# Autodesk Inventor assembly: CaseC
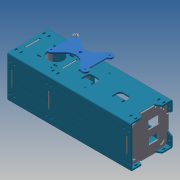
[picture p0: Inventor's stored thumbnail of the model, 180x180]
Saved by Autodesk Inventor 2017 (Build 210142000, 142)
## iProperties
Part Number: CaseC
Material: Genérico
Document SubType Name: Assembly
Designer: Leo
Author: Leo
## Documents named in this file (7)
- C:\Users\FABLAB\Documents\GitHub\actor-re-actor\models\inventor-caja\Case\CaseC.iam
- C:\Users\FABLAB\Documents\GitHub\actor-re-actor\models\inventor-caja\Case\Protector.ipt
- C:\Users\FABLAB\Documents\GitHub\actor-re-actor\models\inventor-caja\Case\Pieza4.ipt
- C:\Users\FABLAB\Documents\GitHub\actor-re-actor\models\inventor-caja\Case\Pliegue Principal.ipt
- C:\Users\FABLAB\Documents\GitHub\actor-re-actor\models\inventor-caja\Case\refuerzo interior.ipt
- C:\Users\FABLAB\Documents\GitHub\actor-re-actor\models\inventor-caja\Case\Tapa Enchufes b.ipt
- C:\Users\FABLAB\Documents\GitHub\actor-re-actor\models\inventor-caja\Case\CaseC\Design Accelerator\Conexión por perno1.iam
## Components (6 placed, 6 different names)
1. Pliegue Principal:1 — Nivelación:8, Nivelación:10, Nivelación:11, Nivelación:13, Nivelación:15, Coincidencia:3
2. Protector:1 — Nivelación:1, Nivelación:2, Nivelación:3, Coincidencia:4, Coincidencia:5
3. Tapa Enchufes b:1 — Nivelación:8, Nivelación:9, Nivelación:10
4. Pieza4:1 — Nivelación:11, Nivelación:12, Nivelación:13
5. refuerzo interior:1 — Nivelación:14, Nivelación:15, Coincidencia:3
6. Conexión por perno:1 [sub-assembly] — Coincidencia:4, Coincidencia:5
## Relationships (14: Flush 11, Mate 3)
- Nivelación:1 [Flush] (45 mm): Protector:1
- Nivelación:2 [Flush]: Protector:1
- Nivelación:3 [Flush]: Protector:1
- Nivelación:8 [Flush]: Pliegue Principal:1 ↔ Tapa Enchufes b:1
- Nivelación:9 [Flush]: Tapa Enchufes b:1
- Nivelación:10 [Flush]: Pliegue Principal:1 ↔ Tapa Enchufes b:1
- Nivelación:11 [Flush]: Pliegue Principal:1 ↔ Pieza4:1
- Nivelación:12 [Flush]: Pieza4:1
- Nivelación:13 [Flush]: Pliegue Principal:1 ↔ Pieza4:1
- Nivelación:14 [Flush]: refuerzo interior:1
- Nivelación:15 [Flush]: Pliegue Principal:1 ↔ refuerzo interior:1
- Coincidencia:3 [Mate]: Pliegue Principal:1 ↔ refuerzo interior:1
- Coincidencia:4 [Mate]: Protector:1 ↔ Conexión por perno:1
- Coincidencia:5 [Mate]: Protector:1 ↔ Conexión por perno:1
